# Autodesk Inventor assembly: HbSocketU03
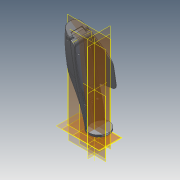
[picture p0: Inventor's stored thumbnail of the model, 180x180]
Saved by Autodesk Inventor 2015 SP1 (Build 190203100, 203)
## iProperties
Created: 2015-08-03
Part Number: HbSocketU03
Document SubType Name: Assembly
Designer: Yamaura
Author: Yamaura
## Documents named in this file (13)
- C:\Users\Yamaura\Documents\GitHub\HACKberry\HACKberry-hardware\3D\Inventor\Parts\HbSocketU03.iam
- C:\Users\Yamaura\Documents\GitHub\HACKberry\HACKberry-hardware\3D\Inventor\Parts\HbMainFrameB03.ipt
- C:\Users\Yamaura\Documents\GitHub\HACKberry\HACKberry-hardware\3D\Inventor\Parts\HbMainFrameA03.ipt
- C:\Users\Yamaura\Documents\GitHub\HACKberry\HACKberry-hardware\3D\Inventor\Parts\HbBatteryLockKnob01.ipt
- C:\Users\Yamaura\Documents\GitHub\HACKberry\HACKberry-hardware\3D\Inventor\Parts\HbBatteryDoorB03.ipt
- C:\Users\Yamaura\Documents\GitHub\HACKberry\HACKberry-hardware\3D\Inventor\Parts\HbBatteryDoorA03.ipt
- C:\Users\Yamaura\Documents\GitHub\HACKberry\HACKberry-hardware\3D\Inventor\Parts\HbBatteryDoorShaft03.ipt
- C:\Users\Yamaura\Documents\GitHub\HACKberry\HACKberry-hardware\3D\Inventor\Parts\HbBatteryDoorShaftStopper03.ipt
- C:\Users\Yamaura\Documents\GitHub\HACKberry\HACKberry-hardware\3D\Inventor\Parts\HbBatteryPcb01.ipt
- C:\Users\Yamaura\Documents\GitHub\HACKberry\HACKberry-hardware\3D\Inventor\Parts\VN-3-1.ipt
- C:\Users\Yamaura\Documents\GitHub\HACKberry\HACKberry-hardware\3D\Inventor\Parts\DMW-BLF19.ipt
- C:\Users\Yamaura\Documents\GitHub\HACKberry\HACKberry-hardware\3D\Inventor\Parts\HbBatteryCase04.ipt
- C:\Users\Yamaura\Documents\GitHub\HACKberry\HACKberry-hardware\3D\Inventor\Parts\flatScrewM2L4PHI3.3T1.3.ipt
## Components (16 placed, 12 different names)
1. HbMainFrameA03:1 — フラッシュ:1, フラッシュ:3, メイト:1, メイト:2, メイト:3, メイト:8
2. HbMainFrameB03:1 — メイト:2, メイト:3, メイト:7, メイト:8, 角度:1, メイト:10, メイト:11, メイト:15, メイト:17, メイト:20, メイト:21, 角度:4, メイト:29, メイト:30, メイト:31, メイト:34, メイト:35, メイト:36, メイト:37
3. HbBatteryLockKnob01:1 — メイト:7, 角度:1
4. HbBatteryDoorB03:1 — メイト:10, メイト:11, メイト:12, メイト:13, メイト:14, メイト:16
5. HbBatteryDoorA03:1 — メイト:12, メイト:13, メイト:14, 角度:2
6. HbBatteryDoorShaft03:1 — メイト:15, メイト:16, 角度:3, メイト:18, メイト:19
7. HbBatteryDoorShaftStopper03:1 — メイト:17, 角度:3, メイト:18, メイト:19
8. HbBatteryPcb01:1 — メイト:20, メイト:21, 角度:4, メイト:24, メイト:25, メイト:32, メイト:33
9. VN-3-1:1 — メイト:25, メイト:33
10. VN-3-1:2 — メイト:24, メイト:32
11. DMW-BLF19:1
12. HbBatteryCase04:1 — メイト:29, メイト:30, メイト:31, フラッシュ:4, フラッシュ:5, フラッシュ:6, フラッシュ:7
13. flatScrewM2L4PHI3.3T1.3:1 — フラッシュ:4, メイト:34
14. flatScrewM2L4PHI3.3T1.3:4 — フラッシュ:5, メイト:35
15. flatScrewM2L4PHI3.3T1.3:5 — フラッシュ:6, メイト:37
16. flatScrewM2L4PHI3.3T1.3:6 — フラッシュ:7, メイト:36
## Relationships (38: Mate 28, Flush 6, Angle 4)
- フラッシュ:1 [Flush]: HbMainFrameA03:1
- フラッシュ:3 [Flush]: HbMainFrameA03:1
- メイト:1 [Mate]: HbMainFrameA03:1
- メイト:2 [Mate]: HbMainFrameA03:1 ↔ HbMainFrameB03:1
- メイト:3 [Mate]: HbMainFrameA03:1 ↔ HbMainFrameB03:1
- メイト:7 [Mate]: HbMainFrameB03:1 ↔ HbBatteryLockKnob01:1
- メイト:8 [Mate]: HbMainFrameA03:1 ↔ HbMainFrameB03:1
- 角度:1 [Angle] (180 deg): HbMainFrameB03:1 ↔ HbBatteryLockKnob01:1
- メイト:10 [Mate]: HbMainFrameB03:1 ↔ HbBatteryDoorB03:1
- メイト:11 [Mate] (0.3 mm): HbMainFrameB03:1 ↔ HbBatteryDoorB03:1
- メイト:12 [Mate]: HbBatteryDoorB03:1 ↔ HbBatteryDoorA03:1
- メイト:13 [Mate]: HbBatteryDoorB03:1 ↔ HbBatteryDoorA03:1
- メイト:14 [Mate]: HbBatteryDoorB03:1 ↔ HbBatteryDoorA03:1
- 角度:2 [Angle] (0 deg): HbBatteryDoorA03:1
- メイト:15 [Mate]: HbMainFrameB03:1 ↔ HbBatteryDoorShaft03:1
- メイト:16 [Mate] (0.2 mm): HbBatteryDoorB03:1 ↔ HbBatteryDoorShaft03:1
- メイト:17 [Mate]: HbMainFrameB03:1 ↔ HbBatteryDoorShaftStopper03:1
- 角度:3 [Angle] (0 deg): HbBatteryDoorShaft03:1 ↔ HbBatteryDoorShaftStopper03:1
- メイト:18 [Mate]: HbBatteryDoorShaft03:1 ↔ HbBatteryDoorShaftStopper03:1
- メイト:19 [Mate]: HbBatteryDoorShaft03:1 ↔ HbBatteryDoorShaftStopper03:1
- メイト:20 [Mate]: HbMainFrameB03:1 ↔ HbBatteryPcb01:1
- メイト:21 [Mate]: HbMainFrameB03:1 ↔ HbBatteryPcb01:1
- 角度:4 [Angle] (180 deg): HbMainFrameB03:1 ↔ HbBatteryPcb01:1
- メイト:24 [Mate]: HbBatteryPcb01:1 ↔ VN-3-1:2
- メイト:25 [Mate]: HbBatteryPcb01:1 ↔ VN-3-1:1
- メイト:29 [Mate]: HbMainFrameB03:1 ↔ HbBatteryCase04:1
- メイト:30 [Mate]: HbMainFrameB03:1 ↔ HbBatteryCase04:1
- メイト:31 [Mate]: HbMainFrameB03:1 ↔ HbBatteryCase04:1
- メイト:32 [Mate]: HbBatteryPcb01:1 ↔ VN-3-1:2
- メイト:33 [Mate]: HbBatteryPcb01:1 ↔ VN-3-1:1
- フラッシュ:4 [Flush]: HbBatteryCase04:1 ↔ flatScrewM2L4PHI3.3T1.3:1
- メイト:34 [Mate]: HbMainFrameB03:1 ↔ flatScrewM2L4PHI3.3T1.3:1
- フラッシュ:5 [Flush]: HbBatteryCase04:1 ↔ flatScrewM2L4PHI3.3T1.3:4
- メイト:35 [Mate]: HbMainFrameB03:1 ↔ flatScrewM2L4PHI3.3T1.3:4
- フラッシュ:6 [Flush]: HbBatteryCase04:1 ↔ flatScrewM2L4PHI3.3T1.3:5
- フラッシュ:7 [Flush]: HbBatteryCase04:1 ↔ flatScrewM2L4PHI3.3T1.3:6
- メイト:36 [Mate]: HbMainFrameB03:1 ↔ flatScrewM2L4PHI3.3T1.3:6
- メイト:37 [Mate]: HbMainFrameB03:1 ↔ flatScrewM2L4PHI3.3T1.3:5
